# Autodesk Inventor assembly: outer_mirrored
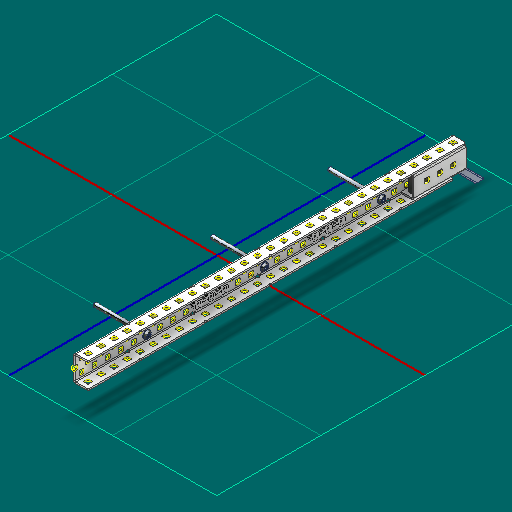
[picture p0: Inventor's stored thumbnail of the model, 512x512]
Saved by Autodesk Inventor 2025 (Build 290162000, 162)
## iProperties
Created: 2024-06-17
Part Number: outer_mirrored
Document SubType Name: Assembly
Designer: Averey Ku
Author: Averey Ku
## Documents named in this file (10)
- C:\Users\avere\vex_robotics_high_stakes\hardware\cad\EARLY_SEASON\chassis\mirrored_parts\outer_mirrored.iam
- C:\Users\avere\vex_robotics_high_stakes\hardware\cad\EARLY_SEASON\chassis\mirrored_parts\C Channel Coupler_mirrored.ipt
- C:\Users\avere\vex_robotics_high_stakes\hardware\cad\VEX-CAD-Inventor\Structure\Hardware\Screw Shoulder Robosource\SScrew Shoulder Smooth 2.000 x .04.ipt
- D:\vex_robotics_high_stakes\hardware\cad\VEX-CAD-Inventor\Structure\Hardware\Screw Shoulder Robosource.ipt
- C:\Users\avere\vex_robotics_high_stakes\hardware\cad\EARLY_SEASON\chassis\mirrored_parts\Bearing Flat Low Profile_mirrored.ipt
- C:\Users\avere\vex_robotics_high_stakes\hardware\cad\EARLY_SEASON\chassis\drivebay\custom_parts\hs_wedge\Shaft HS 2.5 in.ipt
- D:\vex_robotics_high_stakes\hardware\cad\EARLY_SEASON\chassis\drivebay\custom_parts\wedge.ipt
- C:\Users\avere\vex_robotics_high_stakes\hardware\cad\VEX-CAD-Inventor\Structure\Standoff\Standoff .75.ipt
- D:\vex_robotics_high_stakes\hardware\cad\VEX-CAD-Inventor\Structure\Standoff.ipt
- C:\Users\avere\vex_robotics_high_stakes\hardware\cad\EARLY_SEASON\chassis\mirrored_parts\Alu C 1x2x1x29_mirrored.ipt
## Components (9 placed, 6 different names)
1. C Channel Coupler_mirrored:1 — Insert:11, Mate:1, Insert:12
2. SScrew Shoulder Smooth 2.000 x .04:1 — Insert:14
3. Bearing Flat Low Profile_mirrored:1 — Mate:3, Insert:15
4. SScrew Shoulder Smooth 2.000 x .04:2 — Insert:17
5. Bearing Flat Low Profile_mirrored:2 — Mate:2, Insert:16
6. SScrew Shoulder Smooth 2.000 x .04:3 — Insert:18
7. Shaft HS 2.5 in:1 — Angle:1, Insert:13
8. Standoff .75:1 — Insert:11
9. Alu C 1x2x1x29_mirrored:1 — Mate:3, Mate:2, Insert:18, Insert:17, Insert:16, Insert:15, Insert:14, Angle:1, Insert:13, Mate:1, Insert:12
## Relationships (12: Insert 8, Mate 3, Angle 1)
- Insert:11: C Channel Coupler_mirrored:1 ↔ Standoff .75:1
- Mate:3: Bearing Flat Low Profile_mirrored:1 ↔ Alu C 1x2x1x29_mirrored:1
- Mate:2: Bearing Flat Low Profile_mirrored:2 ↔ Alu C 1x2x1x29_mirrored:1
- Insert:18: SScrew Shoulder Smooth 2.000 x .04:3 ↔ Alu C 1x2x1x29_mirrored:1
- Insert:17: SScrew Shoulder Smooth 2.000 x .04:2 ↔ Alu C 1x2x1x29_mirrored:1
- Insert:16: Bearing Flat Low Profile_mirrored:2 ↔ Alu C 1x2x1x29_mirrored:1
- Insert:15: Bearing Flat Low Profile_mirrored:1 ↔ Alu C 1x2x1x29_mirrored:1
- Insert:14: SScrew Shoulder Smooth 2.000 x .04:1 ↔ Alu C 1x2x1x29_mirrored:1
- Angle:1 (0 deg): Shaft HS 2.5 in:1 ↔ Alu C 1x2x1x29_mirrored:1
- Insert:13: Shaft HS 2.5 in:1 ↔ Alu C 1x2x1x29_mirrored:1
- Mate:1: C Channel Coupler_mirrored:1 ↔ Alu C 1x2x1x29_mirrored:1
- Insert:12: C Channel Coupler_mirrored:1 ↔ Alu C 1x2x1x29_mirrored:1
